# Autodesk Inventor assembly: LPS
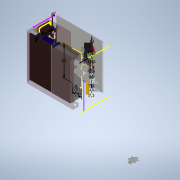
[picture p0: Inventor's stored thumbnail of the model, 180x180]
Saved by Autodesk Inventor 2022 (Build 260153000, 153)
## iProperties
Created: 2024-07-04
Part Number: LPS
Document SubType Name: Assembly
Designer: Капустяник Андрей
Author: Капустяник Андрей
## Documents named in this file (20)
- C:\Users\akapu\OneDrive\Документы\Git\camp2024\LPC_case\LPS.iam
- C:\Users\akapu\OneDrive\Документы\Git\camp2024\LPC_case\power unit.ipt
- C:\Users\akapu\OneDrive\Документы\Git\camp2024\LPC_case\LPS_board.ipt
- C:\Users\akapu\OneDrive\Документы\Git\camp2024\LPC_case\User Library-potenciometro.ipt
- C:\Users\akapu\OneDrive\Документы\Git\camp2024\LPC_case\volt-amp_f2p.ipt
- C:\Users\akapu\OneDrive\Документы\Git\camp2024\LPC_case\volt-amp_f3p.ipt
- C:\Users\akapu\OneDrive\Документы\Git\camp2024\LPC_case\volt-amp_pcb.ipt
- C:\Users\akapu\OneDrive\Документы\Git\camp2024\LPC_case\volt-amp_boitier.ipt
- C:\Users\akapu\OneDrive\Документы\Git\camp2024\LPC_case\LPS_base.ipt
- C:\Users\akapu\OneDrive\Документы\Git\camp2024\LPC_case\interlock_switch_male_wFuse v13.ipt
- C:\Users\akapu\OneDrive\Документы\Git\camp2024\LPC_case\LPS_cap.ipt
- C:\Users\akapu\OneDrive\Документы\Git\camp2024\LPC_case\ALSRobot-LED 8mm.ipt
- C:\Users\akapu\OneDrive\Документы\Git\camp2024\LPC_case\Переключатель сетевой B100G-R SWR41.ipt
- C:\Users\akapu\OneDrive\Документы\Git\camp2024\LPC_case\9.5 MM PUSH BUTTON.ipt
- C:\Users\akapu\OneDrive\Документы\Git\camp2024\LPC_case\led_cap.ipt
- C:\Users\akapu\OneDrive\Документы\Git\camp2024\LPC_case\banana plug.ipt
- C:\Users\akapu\OneDrive\Документы\Git\camp2024\LPC_case\404010 Fan v5.ipt
- C:\Users\akapu\OneDrive\Документы\Git\camp2024\LPC_case\User Library-DS1069-3 CWF-3.ipt
- C:\Users\akapu\OneDrive\Документы\Git\camp2024\LPC_case\User Library-DS1069-2 CWF-2.ipt
- C:\Users\akapu\OneDrive\Документы\Git\camp2024\LPC_case\User Library-640456-2.ipt
## Components (27 placed, 19 different names)
1. power unit:1 — Совмещение:38, Совмещение:39, Совмещение:41, Совмещение:43
2. LPS_board:1 — Совмещение:40, Совмещение:42, Совмещение:43, Совмещение:47, Совмещение:48, Совмещение:49, Совмещение:50, Совмещение:51, Совмещение:52, Совмещение:53, Совмещение:54, Совмещение:56, Совмещение:57
3. volt-amp_f2p:1 — Совмещение:1, Совмещение:2, Совмещение:3
4. volt-amp_f3p:1 — Совмещение:4, Совмещение:5, Совмещение:6
5. volt-amp_pcb:1 — Совмещение:1, Совмещение:2, Совмещение:3, Совмещение:4, Совмещение:5, Совмещение:6, Совмещение:7, Совмещение:8, Совмещение:9
6. volt-amp_boitier:1 — Совмещение:7, Совмещение:8, Совмещение:9, Совмещение:25, Совмещение:26
7. LPS_base:1 — Совмещение:10, Совмещение:37, Совмещение:38, Совмещение:39, Совмещение:40, Совмещение:41, Совмещение:42, Заподлицо:3, Заподлицо:4, Совмещение:44, Совмещение:45
8. interlock_switch_male_wFuse v13:1 — Совмещение:10, Совмещение:37
9. LPS_cap:1 — Совмещение:16, Совмещение:17, Совмещение:21, Совмещение:22, Совмещение:23, Совмещение:24, Совмещение:25, Совмещение:26, Совмещение:29, Совмещение:46
10. User Library-potenciometro:4 — Совмещение:17
11. ALSRobot-LED 8mm:1 — Совмещение:16, Совмещение:21
12. Переключатель сетевой B100G-R SWR41:1 — Совмещение:23, Совмещение:24
13. 9.5 MM PUSH BUTTON:1 — Совмещение:22
14. User Library-potenciometro:7 — Совмещение:29
15. led_cap:1
16. banana plug:1 — Заподлицо:3, Заподлицо:4, Совмещение:44
17. 404010 Fan v5:1 — Совмещение:45, Совмещение:46
18. User Library-DS1069-3 CWF-3:1 — Совмещение:47
19. User Library-DS1069-2 CWF-2:1 — Совмещение:48
20. User Library-640456-2:1 — Совмещение:49
21. User Library-DS1069-2 CWF-2:2 — Совмещение:53
22. User Library-DS1069-2 CWF-2:3 — Совмещение:52
23. User Library-DS1069-3 CWF-3:2 — Совмещение:50
24. User Library-DS1069-3 CWF-3:3 — Совмещение:51
25. User Library-640456-2:2 — Совмещение:54
26. User Library-640456-2:3 — Совмещение:56
27. User Library-640456-2:4 — Совмещение:57
## Relationships (41: Mate 39, Flush 2)
- Совмещение:1 [Mate]: volt-amp_f2p:1 ↔ volt-amp_pcb:1
- Совмещение:2 [Mate]: volt-amp_f2p:1 ↔ volt-amp_pcb:1
- Совмещение:3 [Mate]: volt-amp_f2p:1 ↔ volt-amp_pcb:1
- Совмещение:4 [Mate]: volt-amp_f3p:1 ↔ volt-amp_pcb:1
- Совмещение:5 [Mate]: volt-amp_f3p:1 ↔ volt-amp_pcb:1
- Совмещение:6 [Mate]: volt-amp_f3p:1 ↔ volt-amp_pcb:1
- Совмещение:7 [Mate]: volt-amp_pcb:1 ↔ volt-amp_boitier:1
- Совмещение:8 [Mate]: volt-amp_pcb:1 ↔ volt-amp_boitier:1
- Совмещение:9 [Mate]: volt-amp_pcb:1 ↔ volt-amp_boitier:1
- Совмещение:10 [Mate]: LPS_base:1 ↔ interlock_switch_male_wFuse v13:1
- Совмещение:16 [Mate]: LPS_cap:1 ↔ ALSRobot-LED 8mm:1
- Совмещение:17 [Mate]: LPS_cap:1 ↔ User Library-potenciometro:4
- Совмещение:21 [Mate]: LPS_cap:1 ↔ ALSRobot-LED 8mm:1
- Совмещение:22 [Mate]: LPS_cap:1 ↔ 9.5 MM PUSH BUTTON:1
- Совмещение:23 [Mate]: LPS_cap:1 ↔ Переключатель сетевой B100G-R SWR41:1
- Совмещение:24 [Mate]: LPS_cap:1 ↔ Переключатель сетевой B100G-R SWR41:1
- Совмещение:25 [Mate]: volt-amp_boitier:1 ↔ LPS_cap:1
- Совмещение:26 [Mate]: volt-amp_boitier:1 ↔ LPS_cap:1
- Совмещение:29 [Mate]: LPS_cap:1 ↔ User Library-potenciometro:7
- Совмещение:37 [Mate]: LPS_base:1 ↔ interlock_switch_male_wFuse v13:1
- Совмещение:38 [Mate] (4 mm): power unit:1 ↔ LPS_base:1
- Совмещение:39 [Mate]: power unit:1 ↔ LPS_base:1
- Совмещение:40 [Mate]: LPS_board:1 ↔ LPS_base:1
- Совмещение:41 [Mate] (2 mm): power unit:1 ↔ LPS_base:1
- Совмещение:42 [Mate]: LPS_board:1 ↔ LPS_base:1
- Совмещение:43 [Mate] (5 mm): power unit:1 ↔ LPS_board:1
- Заподлицо:3 [Flush]: LPS_base:1 ↔ banana plug:1
- Заподлицо:4 [Flush]: LPS_base:1 ↔ banana plug:1
- Совмещение:44 [Mate]: LPS_base:1 ↔ banana plug:1
- Совмещение:45 [Mate]: LPS_base:1 ↔ 404010 Fan v5:1
- Совмещение:46 [Mate]: LPS_cap:1 ↔ 404010 Fan v5:1
- Совмещение:47 [Mate]: LPS_board:1 ↔ User Library-DS1069-3 CWF-3:1
- Совмещение:48 [Mate]: LPS_board:1 ↔ User Library-DS1069-2 CWF-2:1
- Совмещение:49 [Mate] (0.5 mm): LPS_board:1 ↔ User Library-640456-2:1
- Совмещение:50 [Mate]: LPS_board:1 ↔ User Library-DS1069-3 CWF-3:2
- Совмещение:51 [Mate]: LPS_board:1 ↔ User Library-DS1069-3 CWF-3:3
- Совмещение:52 [Mate]: LPS_board:1 ↔ User Library-DS1069-2 CWF-2:3
- Совмещение:53 [Mate]: LPS_board:1 ↔ User Library-DS1069-2 CWF-2:2
- Совмещение:54 [Mate] (0.5 mm): LPS_board:1 ↔ User Library-640456-2:2
- Совмещение:56 [Mate] (0.5 mm): LPS_board:1 ↔ User Library-640456-2:3
- Совмещение:57 [Mate] (0.5 mm): LPS_board:1 ↔ User Library-640456-2:4
